# Autodesk Inventor assembly: Chain Drive
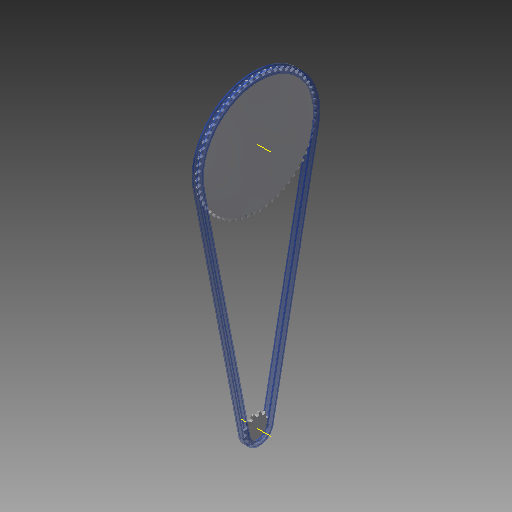
[picture p0: Inventor's stored thumbnail of the model, 512x512]
Saved by Autodesk Inventor 2018.2 (Build 222227000, 227)
## iProperties
Created: 2018-02-07
Part Number: Chain Drive
Document SubType Name: Assembly
Designer: steele
ClientObjectVersion: 1
Author: steele
## Documents named in this file (4)
- D:\snobotics\CAD-Development\robSteele\2018-FRC\Arm\ArmFrameWithMotorAndGears\Design Accelerator\Chain Drive1.iam
- D:\snobotics\CAD-Development\robSteele\2018-FRC\Arm\ArmFrameWithMotorAndGears\Design Accelerator\Roller Chain1.ipt
- D:\snobotics\CAD-Development\robSteele\2018-FRC\Arm\ArmFrameWithMotorAndGears\Design Accelerator\Roller Chain Sprocket11.ipt
- D:\snobotics\CAD-Development\robSteele\2018-FRC\Arm\ArmFrameWithMotorAndGears\Design Accelerator\Roller Chain Sprocket21.ipt
## Components (3 placed, 3 different names)
1. Roller Chain:1 — Flush:1, Mate:1, Mate:2, Flush:2, Mate:3, Mate:4
2. Roller Chain Sprocket1:1 — Flush:1, Mate:1, Mate:2, Rotation:1
3. Roller Chain Sprocket2:1 — Flush:2, Mate:3, Rotation:1, Mate:4
## Relationships (7: Mate 4, Flush 2, RelateRotation 1)
- Flush:1: Roller Chain:1 ↔ Roller Chain Sprocket1:1
- Mate:1: Roller Chain:1 ↔ Roller Chain Sprocket1:1
- Mate:2: Roller Chain:1 ↔ Roller Chain Sprocket1:1
- Flush:2: Roller Chain:1 ↔ Roller Chain Sprocket2:1
- Mate:3: Roller Chain:1 ↔ Roller Chain Sprocket2:1
- Rotation:1 [RelateRotation] (5 ul): Roller Chain Sprocket1:1 ↔ Roller Chain Sprocket2:1
- Mate:4: Roller Chain:1 ↔ Roller Chain Sprocket2:1
